# Autodesk Inventor assembly: Thermostat_bottle_holder
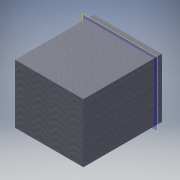
[picture p0: Inventor's stored thumbnail of the model, 180x180]
Saved by Autodesk Inventor 2017 (Build 210142000, 142)
## iProperties
Created: 2016-11-02
Part Number: Thermostat_bottle_holder
Document SubType Name: Assembly
Designer: Camilo
Author: Camilo
## Documents named in this file (3)
- Z:\Github\AgingTests\3D parts\Thermostat bottle holder\Thermostat_bottle_holder.iam
- Z:\Github\AgingTests\3D parts\Thermostat bottle holder\thermostatBath.ipt
- Z:\Github\AgingTests\3D parts\Thermostat bottle holder\bottleHolder.ipt
## Components (2 placed, 2 different names)
1. thermostatBath:1 — Flush:1, Flush:2
2. bottleHolder:1 — Flush:1, Flush:2
## Relationships (2: Flush 2)
- Flush:1: thermostatBath:1 ↔ bottleHolder:1
- Flush:2 (-20 mm): thermostatBath:1 ↔ bottleHolder:1
